# Autodesk Inventor assembly: 조립품1
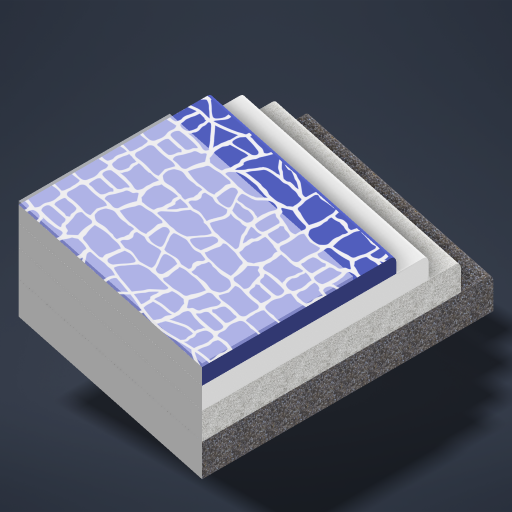
[picture p0: Inventor's stored thumbnail of the model, 512x512]
Saved by Autodesk Inventor 2024 (Build 280153000, 153)
## iProperties
Created: 2024-01-19
Part Number: 조립품1
Document SubType Name: Assembly
Designer: KBU
Author: KBU
## Documents named in this file (3)
- D:\github\Modeling\두원칼라콘크리트\[조립]2번 작업물.iam
- D:\github\Modeling\두원칼라콘크리트\2번 작업물.ipt
- D:\github\Modeling\두원칼라콘크리트\코팅면.ipt
## Components (2 placed, 2 different names)
1. 2번 작업물:1 — 강체:1
2. 코팅면:1 — 강체:1
## Relationships (1: WeldJoint 1)
- 강체:1 [WeldJoint]: 2번 작업물:1 ↔ 코팅면:1
